# Autodesk Inventor assembly: derive_base_plate_v6
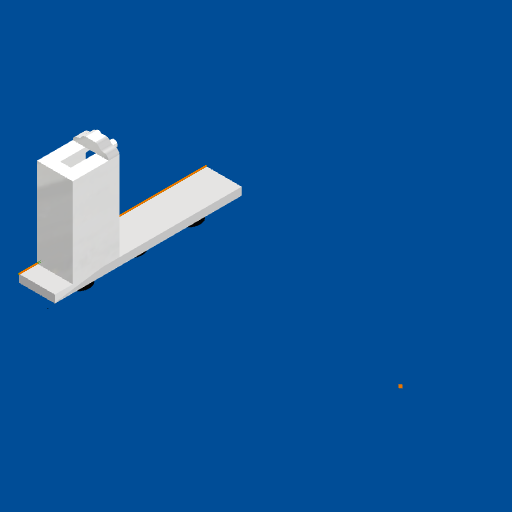
[picture p0: Inventor's stored thumbnail of the model, 512x512]
Saved by Autodesk Inventor 2026.2 (Build 302298000, 298)
## iProperties
Created: 2026-01-17
Part Number: derive_base_plate_v6
Document SubType Name: Assembly
Designer: Thoma
Author: Thoma
## Documents named in this file (3)
- C:\Users\Thoma\OneDrive\Desktop\dir\telescope_cover\cover\derive_base_plate_v6.iam
- C:\Users\Thoma\OneDrive\Desktop\dir\telescope_cover\cover\base+casing_v1.ipt
- C:\Users\Thoma\OneDrive\Desktop\dir\telescope_cover\cover\Base_Plate_v2.ipt
## Components (2 placed, 2 different names)
1. base+casing_v1:1 — Flush:1, Flush:2, Flush:3
2. Base_Plate_v2:1 — Flush:1, Flush:2, Flush:3
## Relationships (3: Flush 3)
- Flush:1: base+casing_v1:1 ↔ Base_Plate_v2:1
- Flush:2: base+casing_v1:1 ↔ Base_Plate_v2:1
- Flush:3: base+casing_v1:1 ↔ Base_Plate_v2:1
